# Autodesk Inventor assembly: allen key holder
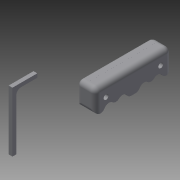
[picture p0: Inventor's stored thumbnail of the model, 180x180]
Saved by Autodesk Inventor 2015 (Build 190159000, 159)
## iProperties
Created: 2014-11-04
Part Number: allen key holder
Document SubType Name: Assembly
Designer: jesse
Author: jesse
## Documents named in this file (4)
- C:\Users\jesse\Desktop\robot\tools\allen key holder.iam
- C:\Users\jesse\Desktop\robot\tools\allen key.ipt
- C:\Users\jesse\Desktop\robot\tools\handle.ipt
- C:\Users\jesse\Desktop\robot\tools\handle1.ipt
## Components (3 placed, 3 different names)
1. allen key:1
2. handle:1 — Mate:1, Mate:2, Mate:3
3. handle1:1 — Mate:1, Mate:2, Mate:3
## Relationships (3: Mate 3)
- Mate:1: handle:1 ↔ handle1:1
- Mate:2: handle:1 ↔ handle1:1
- Mate:3: handle:1 ↔ handle1:1
